# Autodesk Inventor assembly: Overall_Assembly_Rev2
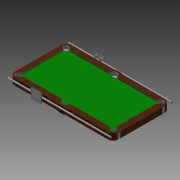
[picture p0: Inventor's stored thumbnail of the model, 180x180]
Saved by Autodesk Inventor 2015 (Build 190159000, 159)
## iProperties
Created: 2016-12-23
Part Number: Overall_Assembly_Rev2
Document SubType Name: Assembly
Designer: Guy
Author: Guy
## Documents named in this file (3)
- C:\Users\Guy\Documents\Fourth Year\Capstone\git\Capstone-Project\doc\CAD\LowLevel_Rev2\Overall_Assembly_Rev2.iam
- C:\Users\Guy\Documents\Fourth Year\Capstone\git\Capstone-Project\doc\CAD\Pool Table\Table_Model.ipt
- C:\Users\Guy\Documents\Fourth Year\Capstone\git\Capstone-Project\doc\CAD\LowLevel_Rev2\X_rail_Assembly_Rev2.iam
## Components (3 placed, 2 different names)
1. Table_Model:1 — Mate:1, Angle:1, Flush:1, Flush:2, Mate:2, Angle:2, Flush:3, Flush:4
2. X_rail_Assembly_Rev2:1 [sub-assembly] — Mate:2, Angle:2, Flush:3, Flush:4, Mate:3
3. X_rail_Assembly_Rev2:2 [sub-assembly] — Mate:1, Angle:1, Flush:1, Flush:2, Mate:3
## Relationships (9: Flush 4, Mate 3, Angle 2)
- Mate:1: Table_Model:1 ↔ X_rail_Assembly_Rev2:2
- Angle:1 (0 deg): Table_Model:1 ↔ X_rail_Assembly_Rev2:2
- Flush:1 (30 mm): Table_Model:1 ↔ X_rail_Assembly_Rev2:2
- Flush:2: Table_Model:1 ↔ X_rail_Assembly_Rev2:2
- Mate:2: Table_Model:1 ↔ X_rail_Assembly_Rev2:1
- Angle:2 (0 deg): Table_Model:1 ↔ X_rail_Assembly_Rev2:1
- Flush:3: Table_Model:1 ↔ X_rail_Assembly_Rev2:1
- Flush:4 (30 mm): Table_Model:1 ↔ X_rail_Assembly_Rev2:1
- Mate:3: X_rail_Assembly_Rev2:1 ↔ X_rail_Assembly_Rev2:2
